# Autodesk Inventor assembly: Tool_Head
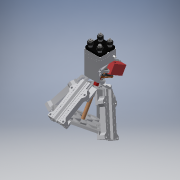
[picture p0: Inventor's stored thumbnail of the model, 180x180]
Saved by Autodesk Inventor 2019 (Build 230136000, 136)
## iProperties
Created: 2021-01-18
Part Number: Tool_Head
Document SubType Name: Assembly
Designer: zhanb
Author: zhanb
## Documents named in this file (18)
- F:\3D Objects\Inventor\Coursework\ECE HyperRail\Tool_Head_Assem.iam
- F:\3D Objects\Inventor\Coursework\ECE HyperRail\Pen_Holder_Assem.iam
- F:\3D Objects\Inventor\Coursework\ECE HyperRail\4-Tool_Lower.ipt
- F:\3D Objects\Inventor\Coursework\ECE HyperRail\4-Tool_Upper.ipt
- F:\3D Objects\Inventor\Coursework\ECE HyperRail\Gantry\Mini V Gantry Kit.iam
- F:\3D Objects\Inventor\Coursework\ECE HyperRail\Gantry_Mount_Rail.ipt
- F:\3D Objects\Inventor\Coursework\ECE HyperRail\Gantry_Mount.ipt
- F:\3D Objects\Inventor\Coursework\ECE HyperRail\Stock Parts\Release_Pin.ipt
- F:\3D Objects\Inventor\Coursework\ECE HyperRail\Stock Parts\.375_Dowel.ipt
- F:\3D Objects\Inventor\Coursework\ECE HyperRail\Stock Parts\.375ID_FlngBearing.ipt
- F:\3D Objects\Inventor\Coursework\ECE HyperRail\Stock Parts\.375_Collar.ipt
- F:\3D Objects\Inventor\Coursework\ECE HyperRail\Stock Parts\Servo_Block.ipt
- F:\3D Objects\Inventor\Coursework\ECE HyperRail\Stock Parts\Servo_Bracket.ipt
- F:\3D Objects\Inventor\Coursework\ECE HyperRail\1.0OD_Pulley.ipt
- F:\3D Objects\Inventor\Coursework\ECE HyperRail\0.75OD_Pulley.ipt
- F:\3D Objects\Inventor\Coursework\ECE HyperRail\0.375ID_0.125_Spacer.ipt
- F:\3D Objects\Inventor\Coursework\ECE HyperRail\Pulley_Belt.ipt
- F:\3D Objects\Inventor\Coursework\ECE HyperRail\0.375ID_0.2_Spacer.ipt
## Components (24 placed, 17 different names)
1. Mini V Gantry Kit:1 [sub-assembly] — Mate:11, Mate:12, Flush:14, Mate:13, Mate:14, Mate:15
2. Gantry_Mount_Rail:1 — Mate:13, Mate:14, Mate:15, Mate:16, Mate:17, Flush:17
3. Gantry_Mount:1 — Mate:16, Mate:20, Mate:17, Mate:18, Mate:25, Mate:32, Mate:33, Angle:5, Mate:39, Mate:40, Flush:17, Angle:6
4. 4-Tool_Upper:1 — Mate:2, Flush:9, Flush:10, Flush:11, Flush:12, Mate:3, Mate:20, Mate:54, Mate:55, Angle:7, Angle:6
5. 4-Tool_Lower:1 — Flush:9, Flush:10, Flush:11, Flush:12, Mate:4, Flush:15, Mate:27
6. Release_Pin:1 — Mate:18
7. .375_Dowel:1 — Flush:15, Mate:26, Mate:28, Mate:30, Mate:31, Mate:33, Mate:43, Mate:48, Mate:49, Mate:51, Mate:53, Mate:55
8. .375ID_FlngBearing:1 — Mate:25, Mate:26, Mate:44, Mate:47
9. .375ID_FlngBearing:2 — Mate:29, Mate:31, Mate:32, Mate:52
10. .375_Collar:1 — Mate:27, Mate:28
11. .375_Collar:2 — Mate:29, Mate:30
12. Servo_Block:1 — Angle:5, Mate:35, Mate:36, Mate:37, Mate:42
13. Servo_Bracket:1 — Mate:35, Mate:36, Mate:37, Mate:39, Mate:40
14. 1.0OD_Pulley:1 — Flush:16, Mate:49, Mate:50, Angle:7
15. 0.75OD_Pulley:1 — Mate:42, Flush:16, Flush:18
16. 0.375ID_0.2_Spacer:2 — Mate:43, Mate:44
17. 0.375ID_0.2_Spacer:3 — Mate:47, Mate:48, Mate:50
18. 0.375ID_0.2_Spacer:1 — Mate:53, Mate:54
19. 0.375ID_0.125_Spacer:1 — Mate:51, Mate:52
20. Pulley_Belt:1 — Flush:18
21. Pen_Holder_Assem:1 [sub-assembly] — Mate:2, Mate:3, Mate:4
22. Pen_Holder_Assem:2 [sub-assembly]
23. Pen_Holder_Assem:3 [sub-assembly]
24. Pen_Holder_Assem:4 [sub-assembly]
## Component patterns: (4 elements, first: Pen_Holder_Assem:1)
## Relationships (50: Mate 38, Flush 9, Angle 3)
- Mate:2: 4-Tool_Upper:1 ↔ Pen_Holder_Assem:1
- Flush:9: 4-Tool_Upper:1 ↔ 4-Tool_Lower:1
- Flush:10: 4-Tool_Upper:1 ↔ 4-Tool_Lower:1
- Flush:11: 4-Tool_Upper:1 ↔ 4-Tool_Lower:1
- Flush:12: 4-Tool_Upper:1 ↔ 4-Tool_Lower:1
- Mate:3: 4-Tool_Upper:1 ↔ Pen_Holder_Assem:1
- Mate:4: 4-Tool_Lower:1 ↔ Pen_Holder_Assem:1
- Mate:11: Mini V Gantry Kit:1
- Mate:12: Mini V Gantry Kit:1
- Flush:14: Mini V Gantry Kit:1
- Mate:13: Mini V Gantry Kit:1 ↔ Gantry_Mount_Rail:1
- Mate:14: Mini V Gantry Kit:1 ↔ Gantry_Mount_Rail:1
- Mate:15: Mini V Gantry Kit:1 ↔ Gantry_Mount_Rail:1
- Mate:16 (0.1984 mm): Gantry_Mount_Rail:1 ↔ Gantry_Mount:1
- Mate:20 (11.938 mm): Gantry_Mount:1 ↔ 4-Tool_Upper:1
- Mate:17: Gantry_Mount_Rail:1 ↔ Gantry_Mount:1
- Mate:18: Gantry_Mount:1 ↔ Release_Pin:1
- Flush:15 (-9.525 mm): 4-Tool_Lower:1 ↔ .375_Dowel:1
- Mate:25: Gantry_Mount:1 ↔ .375ID_FlngBearing:1
- Mate:26: .375_Dowel:1 ↔ .375ID_FlngBearing:1
- Mate:27: 4-Tool_Lower:1 ↔ .375_Collar:1
- Mate:28: .375_Dowel:1 ↔ .375_Collar:1
- Mate:29: .375ID_FlngBearing:2 ↔ .375_Collar:2
- Mate:30: .375_Dowel:1 ↔ .375_Collar:2
- Mate:31: .375_Dowel:1 ↔ .375ID_FlngBearing:2
- Mate:32: Gantry_Mount:1 ↔ .375ID_FlngBearing:2
- Mate:33: Gantry_Mount:1 ↔ .375_Dowel:1
- Angle:5 (0 deg): Gantry_Mount:1 ↔ Servo_Block:1
- Mate:35: Servo_Block:1 ↔ Servo_Bracket:1
- Mate:36: Servo_Block:1 ↔ Servo_Bracket:1
- Mate:37: Servo_Block:1 ↔ Servo_Bracket:1
- Mate:39: Gantry_Mount:1 ↔ Servo_Bracket:1
- Mate:40: Gantry_Mount:1 ↔ Servo_Bracket:1
- Mate:42: Servo_Block:1 ↔ 0.75OD_Pulley:1
- Mate:43: .375_Dowel:1 ↔ 0.375ID_0.2_Spacer:2
- Mate:44: .375ID_FlngBearing:1 ↔ 0.375ID_0.2_Spacer:2
- Mate:47: .375ID_FlngBearing:1 ↔ 0.375ID_0.2_Spacer:3
- Mate:48: .375_Dowel:1 ↔ 0.375ID_0.2_Spacer:3
- Flush:16: 1.0OD_Pulley:1 ↔ 0.75OD_Pulley:1
- Mate:49: .375_Dowel:1 ↔ 1.0OD_Pulley:1
- Mate:50 (0.254 mm): 1.0OD_Pulley:1 ↔ 0.375ID_0.2_Spacer:3
- Mate:51: .375_Dowel:1 ↔ 0.375ID_0.125_Spacer:1
- Mate:52: .375ID_FlngBearing:2 ↔ 0.375ID_0.125_Spacer:1
- Flush:17: Gantry_Mount_Rail:1 ↔ Gantry_Mount:1
- Flush:18: 0.75OD_Pulley:1 ↔ Pulley_Belt:1
- Mate:53: .375_Dowel:1 ↔ 0.375ID_0.2_Spacer:1
- Mate:54: 4-Tool_Upper:1 ↔ 0.375ID_0.2_Spacer:1
- Mate:55: 4-Tool_Upper:1 ↔ .375_Dowel:1
- Angle:7 (0 deg): 4-Tool_Upper:1 ↔ 1.0OD_Pulley:1
- Angle:6 (0 deg): Gantry_Mount:1 ↔ 4-Tool_Upper:1
